# Autodesk Inventor assembly: Actuator 1.6
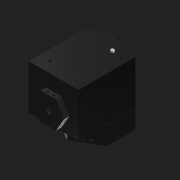
[picture p0: Inventor's stored thumbnail of the model, 180x180]
Saved by Autodesk Inventor 2017 (Build 210142000, 142)
## iProperties
Created: 2019-09-19
Part Number: Actuator 1.6
Document SubType Name: Assembly
Designer: Dell
Author: Dell
## Documents named in this file (8)
- C:\Users\Dell\Documents\GitHub\tr2\Actuator 1.6\Actuator 1.6.iam
- C:\Users\Dell\Documents\GitHub\tr2\Actuator 1.6\AC01.ipt
- C:\Users\Dell\Documents\GitHub\tr2\Actuator 1.6\AC02.ipt
- C:\Users\Dell\Documents\GitHub\tr2\Actuator 1.6\AC03.ipt
- C:\Users\Dell\Documents\GitHub\tr2\Actuator 1.6\AC05.ipt
- C:\Users\Dell\Documents\GitHub\tr2\Actuator 1.6\SEA Gearbox.iam
- C:\Users\Dell\Documents\GitHub\tr2\Actuator 1.6\Slewing.iam
- C:\Users\Dell\Documents\GitHub\tr2\Actuator 1.6\TSINY TS-42GZ495.ipt
## Components (7 placed, 7 different names)
1. AC01:1 — Mate:1, Mate:2, Mate:3, Mate:4, Mate:5, Mate:9, Mate:11, Mate:19
2. AC02:1 — Mate:9, Mate:11, Mate:12, Mate:14, Mate:15, Mate:16, Mate:17, Mate:18, Mate:19
3. AC03:1 — Mate:16, Mate:17, Mate:18
4. AC05:1 — Mate:6, Mate:7, Mate:8
5. SEA Gearbox:1 [sub-assembly] — Mate:1, Mate:2
6. Slewing:1 [sub-assembly] — Mate:3, Mate:4, Mate:5, Mate:6, Mate:7, Mate:8
7. TSINY TS-42GZ495:1 — Mate:12, Mate:14, Mate:15
## Relationships (17: Mate 17)
- Mate:1: AC01:1 ↔ SEA Gearbox:1
- Mate:2: AC01:1 ↔ SEA Gearbox:1
- Mate:3: AC01:1 ↔ Slewing:1
- Mate:4: AC01:1 ↔ Slewing:1
- Mate:5: AC01:1 ↔ Slewing:1
- Mate:6: AC05:1 ↔ Slewing:1
- Mate:7: AC05:1 ↔ Slewing:1
- Mate:8: AC05:1 ↔ Slewing:1
- Mate:9: AC01:1 ↔ AC02:1
- Mate:11: AC01:1 ↔ AC02:1
- Mate:12: AC02:1 ↔ TSINY TS-42GZ495:1
- Mate:14: AC02:1 ↔ TSINY TS-42GZ495:1
- Mate:15: AC02:1 ↔ TSINY TS-42GZ495:1
- Mate:16: AC02:1 ↔ AC03:1
- Mate:17: AC02:1 ↔ AC03:1
- Mate:18: AC02:1 ↔ AC03:1
- Mate:19: AC01:1 ↔ AC02:1
